# Autodesk Inventor assembly: backplane
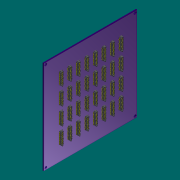
[picture p0: Inventor's stored thumbnail of the model, 180x180]
Saved by Autodesk Inventor 2016 (Build 200138000, 138)
## iProperties
Created: 2015-12-22
Part Number: backplane
Description: for SolidWorks
Document SubType Name: Assembly
Designer: sawai
Authority: Unknown
Sending System: Diptrace
Preprocessor: Open CASCADE STEP processor 6.6
Title: C:\Users\sawai\Desktop\backplane.step
Author: sawai
## Documents named in this file (4)
- C:\Users\sawaiz\oneDrive\projects\modularRICHBackplane\cad\backplane.iam
- C:\Users\sawaiz\oneDrive\projects\modularRICHBackplane\cad\backplane.ipt
- C:\Users\sawaiz\oneDrive\projects\modularRICHBackplane\cad\connectors\SS4-40-3.00-L-D\SS4-40-3_00-L-D.iam
- C:\Users\sawaiz\oneDrive\projects\modularRICHBackplane\cad\connectors\ST4-40-1.00-L-D-P-TR\ST4-40-1_00-L-D-P-TR.iam
## Components (65 placed, 3 different names)
1. backplane:1 — Mate:1, Angle:1, Mate:2, Angle:2
2. SS4-40-3_00-L-D:1 [sub-assembly] — Mate:1, Angle:1
3. SS4-40-3_00-L-D:2 [sub-assembly]
4. SS4-40-3_00-L-D:3 [sub-assembly]
5. SS4-40-3_00-L-D:4 [sub-assembly]
6. SS4-40-3_00-L-D:5 [sub-assembly]
7. SS4-40-3_00-L-D:6 [sub-assembly]
8. SS4-40-3_00-L-D:7 [sub-assembly]
9. SS4-40-3_00-L-D:8 [sub-assembly]
10. SS4-40-3_00-L-D:9 [sub-assembly]
11. SS4-40-3_00-L-D:10 [sub-assembly]
12. SS4-40-3_00-L-D:11 [sub-assembly]
13. SS4-40-3_00-L-D:12 [sub-assembly]
14. SS4-40-3_00-L-D:13 [sub-assembly]
15. SS4-40-3_00-L-D:14 [sub-assembly]
16. SS4-40-3_00-L-D:15 [sub-assembly]
17. SS4-40-3_00-L-D:16 [sub-assembly]
18. SS4-40-3_00-L-D:17 [sub-assembly]
19. SS4-40-3_00-L-D:18 [sub-assembly]
20. SS4-40-3_00-L-D:19 [sub-assembly]
21. SS4-40-3_00-L-D:20 [sub-assembly]
22. SS4-40-3_00-L-D:21 [sub-assembly]
23. SS4-40-3_00-L-D:22 [sub-assembly]
24. SS4-40-3_00-L-D:23 [sub-assembly]
25. SS4-40-3_00-L-D:24 [sub-assembly]
26. SS4-40-3_00-L-D:25 [sub-assembly]
27. SS4-40-3_00-L-D:26 [sub-assembly]
28. SS4-40-3_00-L-D:27 [sub-assembly]
29. SS4-40-3_00-L-D:28 [sub-assembly]
30. SS4-40-3_00-L-D:29 [sub-assembly]
31. SS4-40-3_00-L-D:30 [sub-assembly]
32. SS4-40-3_00-L-D:31 [sub-assembly]
33. SS4-40-3_00-L-D:32 [sub-assembly]
34. ST4-40-1_00-L-D-P-TR:1 [sub-assembly] — Mate:2, Angle:2
35. ST4-40-1_00-L-D-P-TR:2 [sub-assembly]
36. ST4-40-1_00-L-D-P-TR:3 [sub-assembly]
37. ST4-40-1_00-L-D-P-TR:4 [sub-assembly]
38. ST4-40-1_00-L-D-P-TR:5 [sub-assembly]
39. ST4-40-1_00-L-D-P-TR:6 [sub-assembly]
40. ST4-40-1_00-L-D-P-TR:7 [sub-assembly]
41. ST4-40-1_00-L-D-P-TR:8 [sub-assembly]
42. ST4-40-1_00-L-D-P-TR:9 [sub-assembly]
43. ST4-40-1_00-L-D-P-TR:10 [sub-assembly]
44. ST4-40-1_00-L-D-P-TR:11 [sub-assembly]
45. ST4-40-1_00-L-D-P-TR:12 [sub-assembly]
46. ST4-40-1_00-L-D-P-TR:13 [sub-assembly]
47. ST4-40-1_00-L-D-P-TR:14 [sub-assembly]
48. ST4-40-1_00-L-D-P-TR:15 [sub-assembly]
49. ST4-40-1_00-L-D-P-TR:16 [sub-assembly]
50. ST4-40-1_00-L-D-P-TR:17 [sub-assembly]
51. ST4-40-1_00-L-D-P-TR:18 [sub-assembly]
52. ST4-40-1_00-L-D-P-TR:19 [sub-assembly]
53. ST4-40-1_00-L-D-P-TR:20 [sub-assembly]
54. ST4-40-1_00-L-D-P-TR:21 [sub-assembly]
55. ST4-40-1_00-L-D-P-TR:22 [sub-assembly]
56. ST4-40-1_00-L-D-P-TR:23 [sub-assembly]
57. ST4-40-1_00-L-D-P-TR:24 [sub-assembly]
58. ST4-40-1_00-L-D-P-TR:25 [sub-assembly]
59. ST4-40-1_00-L-D-P-TR:26 [sub-assembly]
60. ST4-40-1_00-L-D-P-TR:27 [sub-assembly]
61. ST4-40-1_00-L-D-P-TR:28 [sub-assembly]
62. ST4-40-1_00-L-D-P-TR:29 [sub-assembly]
63. ST4-40-1_00-L-D-P-TR:30 [sub-assembly]
64. ST4-40-1_00-L-D-P-TR:31 [sub-assembly]
65. ST4-40-1_00-L-D-P-TR:32 [sub-assembly]
## Component patterns: (32 elements, first: SS4-40-3_00-L-D:1), (32 elements, first: ST4-40-1_00-L-D-P-TR:1)
## Relationships (4: Mate 2, Angle 2)
- Mate:1: backplane:1 ↔ SS4-40-3_00-L-D:1
- Angle:1 (0 deg): backplane:1 ↔ SS4-40-3_00-L-D:1
- Mate:2: backplane:1 ↔ ST4-40-1_00-L-D-P-TR:1
- Angle:2 (0 deg): backplane:1 ↔ ST4-40-1_00-L-D-P-TR:1
